# Autodesk Inventor assembly: Body
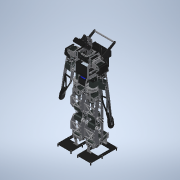
[picture p0: Inventor's stored thumbnail of the model, 180x180]
Saved by Autodesk Inventor 2020.4 (Build 244396000, 396)
## iProperties
Created: 2021-09-30
Part Number: Body
Document SubType Name: Assembly
Designer: Masato Kubotera
Mass: 4468.65 g
Surface Area: 13553.6 cm^2
Volume: 2294.33 cm^3
Density: 1.94769 g/cm^3
Author: Masato Kubotera
## Documents named in this file (4)
- C:\Users\Masato\Documents\Inventor\CIT Brains_Inventor\OpenPlatform_ver3_0\Body.iam
- C:\Users\Masato\Documents\Inventor\CIT Brains_Inventor\OpenPlatform_ver3_0\UpperBody\UpperBody.iam
- C:\Users\Masato\Documents\Inventor\CIT Brains_Inventor\OpenPlatform_ver3_0\LowerBody\LowerBody.iam
- C:\Users\Masato\Documents\Inventor\CIT Brains_Inventor\OpenPlatform_ver3_0\LowerBody\LowerBody_MIR.iam
## Components (3 placed, 3 different names)
1. UpperBody:1 [sub-assembly] — 挿入:1, 挿入:2, フラッシュ:1, フラッシュ:2
2. LowerBody:1 [sub-assembly] — 挿入:1, メイト:1
3. LowerBody_MIR:1 [sub-assembly] — 挿入:2
## Relationships (5: Insert 2, Flush 2, Mate 1)
- 挿入:1 [Insert]: UpperBody:1 ↔ LowerBody:1
- 挿入:2 [Insert]: UpperBody:1 ↔ LowerBody_MIR:1
- フラッシュ:1 [Flush] (-12 mm): UpperBody:1
- メイト:1 [Mate]: LowerBody:1
- フラッシュ:2 [Flush] (-60 mm): UpperBody:1
